# Autodesk Inventor assembly: A1-18002-100-00 Line boring skid
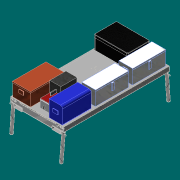
[picture p0: Inventor's stored thumbnail of the model, 180x180]
Saved by Autodesk Inventor 2017 (Build 210142000, 142)
## iProperties
Created: 2018-01-23
Part Number: A1-18002-100-00 Line boring skid
Document SubType Name: Assembly
Designer: Graeme_Van_Dongen
Mass: 2.94826e+06 g
Surface Area: 313203 cm^2
Volume: 587682 cm^3
Density: 5.01675 g/cm^3
Author: Graeme_Van_Dongen
## Documents named in this file (43)
- N:\A1 - Projects\A1-18\A1-18002--Alco Line boring skid\A1-18002-100-00 Line boring skid.iam
- N:\A1 - Projects\A1-18\A1-18002--Alco Line boring skid\Aluminum tool box.ipt
- N:\A1 - Projects\A1-18\A1-18002--Alco Line boring skid\Blue tool box.ipt
- N:\A1 - Projects\A1-18\A1-18002--Alco Line boring skid\Jobox tool box.ipt
- N:\A1 - Projects\A1-18\A1-18002--Alco Line boring skid\Pelican case.ipt
- N:\A1 - Projects\A1-18\A1-18002--Alco Line boring skid\2.25 bar x 8ft.ipt
- N:\A1 - Projects\A1-18\A1-18002--Alco Line boring skid\2.25 bar x 7ft.ipt
- N:\A1 - Projects\A1-18\A1-18002--Alco Line boring skid\2.25 bar x 5ft.ipt
- N:\A1 - Projects\A1-18\A1-18002--Alco Line boring skid\2.25 bar x 3.5ft.ipt
- N:\A1 - Projects\A1-18\A1-18002--Alco Line boring skid\2.25 bar x 3.25ft.ipt
- N:\A1 - Projects\A1-18\A1-18002--Alco Line boring skid\2.25 bar x 3ft.ipt
- N:\A1 - Projects\A1-18\A1-18002--Alco Line boring skid\1.25 bar x 4ft.ipt
- N:\A1 - Projects\A1-18\A1-18002--Alco Line boring skid\1.25 bar x 3ft.ipt
- N:\A1 - Projects\A1-18\A1-18002--Alco Line boring skid\1.25 bar x 2ft.ipt
- N:\A1 - Projects\A1-18\A1-18002--Alco Line boring skid\Welder.ipt
- N:\A1 - Projects\A1-18\A1-18002--Alco Line boring skid\A1-18002-100-20 2.25in x 8ft bar tube.ipt
- N:\A1 - Projects\A1-18\A1-18002--Alco Line boring skid\A1-18002-100-30 2.5in pipe cap.ipt
- ASME B16.11 Cap - Class 3000 2 1/2.ipt
- N:\A1 - Projects\A1-18\A1-18002--Alco Line boring skid\A1-18002-300-00 2.25in bar tube cap.iam
- N:\A1 - Projects\A1-18\A1-18002--Alco Line boring skid\A1-18002-100-21 2.25in x 7ft bar tube.ipt
- N:\A1 - Projects\A1-18\A1-18002--Alco Line boring skid\A1-18002-100-22 2.25in x 5ft bar tube.ipt
- N:\A1 - Projects\A1-18\A1-18002--Alco Line boring skid\A1-18002-100-23 2.25in x 3.5ft bar tube.ipt
- N:\A1 - Projects\A1-18\A1-18002--Alco Line boring skid\A1-18002-100-24 2.25in x 3.25ft bar tube.ipt
- N:\A1 - Projects\A1-18\A1-18002--Alco Line boring skid\A1-18002-100-25 2.25in x 3ft bar tube.ipt
- N:\A1 - Projects\A1-18\A1-18002--Alco Line boring skid\A1-18002-100-31 1.25in x 4ft bar tube.ipt
- N:\A1 - Projects\A1-18\A1-18002--Alco Line boring skid\A1-18002-100-32 1.25in x 3ft bar tube.ipt
- N:\A1 - Projects\A1-18\A1-18002--Alco Line boring skid\A1-18002-100-33 1.25in x 2ft bar tube.ipt
- N:\A1 - Projects\A1-18\A1-18002--Alco Line boring skid\A1-18002-100-36 1.5in pipe cap.ipt
- N:\A1 - Projects\A1-18\A1-18002--Alco Line boring skid\A1-18002-400-00 1.25in bar tube cap.iam
- N:\A1 - Projects\A1-18\A1-18002--Alco Line boring skid\Base frame skeleton.ipt
- N:\A1 - Projects\A1-18\A1-18002--Alco Line boring skid\A1-18002-200-00 Skid leg.iam
- N:\A1 - Projects\A1-18\A1-18002--Alco Line boring skid\Spring latch.ipt
- N:\A1 - Projects\A1-18\A1-18002--Alco Line boring skid\Weld-on hinge #218-109.ipt
- N:\A1 - Projects\A1-18\A1-18002--Alco Line boring skid\A1-18002-100-40 Pocket door plate.ipt
- N:\Inventor\Content Center Files\R2017\en-US\ANSI L(1)\AISC - L 1 x 1 x 1_8 - 32.ipt
- N:\A1 - Projects\A1-18\A1-18002--Alco Line boring skid\A1-18002-150-00 Line boring skid weldment.iam
- N:\Inventor\Content Center Files\R2017\en-US\MS 16624 (3100)\MS 16624 - 0.500S 3100.ipt
- N:\A1 - Projects\A1-18\A1-18002--Alco Line boring skid\Quick release pin.ipt
- N:\A1 - Projects\A1-18\A1-18002--Alco Line boring skid\A1-18002-100-50 Tube cradle - 2.875in.ipt
- N:\A1 - Projects\A1-18\A1-18002--Alco Line boring skid\A1-18002-100-51 Tube cradle - 1.900in.ipt
- N:\A1 - Projects\A1-18\A1-18002--Alco Line boring skid\A1-18002-100-53 Tube stop.ipt
- N:\A1 - Projects\A1-18\A1-18002--Alco Line boring skid\A1-18002-100-52 Tube stop.ipt
- N:\A1 - Projects\A1-18\A1-18002--Alco Line boring skid\A1-18002-100-54 Tube stop.ipt
## Components (101 placed, 41 different names)
1. A1-18002-150-00 Line boring skid weldment:1 [sub-assembly] — Flush:7, Flush:8, Flush:9, Mate:1, Mate:2, Mate:3, Mate:4, Mate:5, Angle:1, Angle:2, Angle:3, Angle:4, Angle:5, Mate:6, Angle:6, Mate:7, Mate:8, Mate:9, Angle:7, Mate:10, Mate:11, Mate:12, Mate:13, Mate:14, Mate:15, Mate:16, Mate:17, Mate:18, Flush:30, Flush:31, Flush:32, Flush:40, Insert:31, Angle:8, Insert:32, Angle:9, Insert:33, Insert:34, Angle:10, Tangent:42, Tangent:43, Angle:12, Angle:13, Angle:14, Angle:15, Angle:16, Angle:17, Angle:18, Angle:19, Angle:20, Angle:21, Angle:22, Angle:23, Angle:24, Angle:25, Angle:26, Angle:27, Angle:28, Angle:29, Angle:30, Angle:31, Angle:32, Angle:33, Angle:34, Angle:35, Angle:36, Angle:37, Mate:49, Mate:50, Mate:52, Mate:54, Mate:57, Mate:59, Mate:61, Mate:63, Mate:66, Mate:69, Mate:72
2. Base frame skeleton:1 — Flush:30, Flush:31, Flush:32
3. Aluminum tool box:1 — Mate:1, Angle:1, Flush:28, Flush:29
4. Aluminum tool box:2 — Mate:2, Angle:2, Flush:28
5. Blue tool box:1 — Mate:3, Angle:3, Flush:29
6. Jobox tool box:1 — Mate:4, Angle:4
7. Pelican case:1 — Mate:5, Angle:5
8. Welder:1 — Mate:6, Angle:6
9. A1-18002-100-40 Pocket door plate:1 — Mate:47, Flush:40, Mate:26, Mate:28, Mate:43, Mate:44, Flush:45, Mate:45, Flush:46, Flush:47, Flush:48, Flush:49, Angle:12
10. Spring latch:1 — Mate:26, Mate:28, Flush:41, Mate:48, Flush:48
11. Spring latch:2 — Flush:41, Mate:48, Flush:49
12. Weld-on hinge #218-109:1 — Flush:42, Mate:43, Tangent:42, Mate:46, Flush:47
13. Weld-on hinge #218-109:2 — Flush:42, Mate:46, Mate:47, Flush:46, Tangent:43
14. ANSI L (Equal angles) L 1 x 1 x 1/8 - 32:1 — Mate:44, Flush:45, Mate:45
15. A1-18002-100-20 2.25in x 8ft bar tube:1 — Insert:1, Insert:2, Mate:7, Angle:7, Flush:10, Flush:18
16. A1-18002-300-00 2.25in bar tube cap:1 [sub-assembly] — Insert:1, Mate:8, Mate:9, Insert:39
17. A1-18002-100-30 2.5in pipe cap:2 — Insert:2, Insert:19, Insert:37, Insert:38
18. A1-18002-100-21 2.25in x 7ft bar tube:1 — Insert:3, Insert:8, Flush:10, Flush:11, Flush:18, Flush:19
19. A1-18002-300-00 2.25in bar tube cap:2 [sub-assembly] — Insert:3, Mate:10, Insert:42
20. A1-18002-100-30 2.5in pipe cap:3 — Insert:8, Insert:20, Insert:40, Insert:41, Mate:51
21. A1-18002-100-22 2.25in x 5ft bar tube:1 — Insert:4, Insert:9, Flush:11, Flush:19, Flush:26, Flush:27
22. A1-18002-300-00 2.25in bar tube cap:3 [sub-assembly] — Insert:4, Mate:11, Insert:45
23. A1-18002-100-30 2.5in pipe cap:4 — Insert:9, Insert:21, Insert:43, Insert:44, Mate:53
24. A1-18002-100-22 2.25in x 5ft bar tube:2 — Insert:28, Insert:30, Flush:26, Flush:27, Flush:20, Flush:12
25. A1-18002-300-00 2.25in bar tube cap:7 [sub-assembly] — Insert:28, Mate:18, Insert:48
26. A1-18002-100-30 2.5in pipe cap:8 — Insert:29, Insert:30, Insert:46, Insert:47, Mate:56
27. A1-18002-100-23 2.25in x 3.5ft bar tube:1 — Insert:5, Insert:10, Flush:12, Flush:13, Flush:20, Flush:21
28. A1-18002-300-00 2.25in bar tube cap:4 [sub-assembly] — Insert:5, Mate:12, Insert:50
29. A1-18002-100-30 2.5in pipe cap:5 — Insert:10, Insert:22, Insert:49, Mate:58
30. A1-18002-100-24 2.25in x 3.25ft bar tube:1 — Insert:6, Insert:11, Flush:13, Flush:14, Flush:21, Flush:22
31. A1-18002-300-00 2.25in bar tube cap:5 [sub-assembly] — Insert:6, Mate:13, Insert:52
32. A1-18002-100-30 2.5in pipe cap:6 — Insert:11, Insert:23, Insert:51, Mate:60
33. A1-18002-100-25 2.25in x 3ft bar tube:1 — Insert:7, Insert:12, Flush:14, Flush:15, Flush:22, Flush:23
34. A1-18002-300-00 2.25in bar tube cap:6 [sub-assembly] — Insert:7, Mate:14, Insert:54
35. A1-18002-100-30 2.5in pipe cap:7 — Insert:12, Insert:24, Insert:53, Mate:62
36. A1-18002-100-31 1.25in x 4ft bar tube:1 — Insert:13, Insert:16, Flush:15, Flush:16, Flush:23, Flush:24
37. A1-18002-400-00 1.25in bar tube cap:1 [sub-assembly] — Insert:13, Mate:15, Insert:57
38. A1-18002-100-36 1.5in pipe cap:1 — Insert:16, Insert:25, Insert:55, Insert:56, Mate:65
39. A1-18002-100-32 1.25in x 3ft bar tube:1 — Insert:14, Insert:17, Flush:16, Flush:17, Flush:24, Flush:25
40. A1-18002-400-00 1.25in bar tube cap:2 [sub-assembly] — Insert:14, Mate:16, Insert:59
41. A1-18002-100-36 1.5in pipe cap:2 — Insert:17, Insert:26, Insert:58, Mate:68
42. A1-18002-100-33 1.25in x 2ft bar tube:1 — Insert:15, Insert:18, Flush:17, Flush:25
43. A1-18002-400-00 1.25in bar tube cap:3 [sub-assembly] — Insert:15, Mate:17, Insert:61
44. A1-18002-100-36 1.5in pipe cap:3 — Insert:18, Insert:27, Insert:60, Mate:71
45. 2.25 bar x 8ft:1 — Insert:19
46. 2.25 bar x 7ft:1 — Insert:20
47. 2.25 bar x 5ft:1 — Insert:29
48. 2.25 bar x 5ft:2 — Insert:21
49. 2.25 bar x 3.5ft:1 — Insert:22
50. 2.25 bar x 3.25ft:1 — Insert:23
51. 2.25 bar x 3ft:1 — Insert:24
52. 1.25 bar x 4ft:1 — Insert:25
53. 1.25 bar x 3ft:1 — Insert:26
54. 1.25 bar x 2ft:1 — Insert:27
55. A1-18002-100-50 Tube cradle - 2.875in:1 — Insert:37, Angle:13, Flush:50
56. A1-18002-100-50 Tube cradle - 2.875in:2 — Insert:38, Angle:14
57. A1-18002-100-50 Tube cradle - 2.875in:3 — Insert:39, Angle:15
58. A1-18002-100-50 Tube cradle - 2.875in:4 — Insert:40, Angle:16, Flush:51
59. A1-18002-100-50 Tube cradle - 2.875in:5 — Insert:41, Angle:17
60. A1-18002-100-50 Tube cradle - 2.875in:6 — Insert:42, Angle:18
61. A1-18002-100-50 Tube cradle - 2.875in:7 — Insert:43, Angle:19, Flush:52
62. A1-18002-100-50 Tube cradle - 2.875in:8 — Insert:44, Angle:20
63. A1-18002-100-50 Tube cradle - 2.875in:9 — Insert:45, Angle:21
64. A1-18002-100-50 Tube cradle - 2.875in:10 — Insert:46, Angle:22, Flush:56
65. A1-18002-100-50 Tube cradle - 2.875in:11 — Insert:47, Angle:23
66. A1-18002-100-50 Tube cradle - 2.875in:12 — Insert:48, Angle:24
67. A1-18002-100-50 Tube cradle - 2.875in:13 — Insert:49, Angle:25, Flush:57
68. A1-18002-100-50 Tube cradle - 2.875in:14 — Insert:50, Angle:26
69. A1-18002-100-50 Tube cradle - 2.875in:15 — Insert:51, Angle:27, Flush:58
70. A1-18002-100-50 Tube cradle - 2.875in:16 — Insert:52, Angle:28
71. A1-18002-100-50 Tube cradle - 2.875in:17 — Insert:53, Angle:29, Flush:59
72. A1-18002-100-50 Tube cradle - 2.875in:18 — Insert:54, Angle:30
73. A1-18002-100-51 Tube cradle - 1.900in:1 — Insert:55, Angle:31, Mate:64
74. A1-18002-100-51 Tube cradle - 1.900in:2 — Insert:56, Angle:32
75. A1-18002-100-51 Tube cradle - 1.900in:3 — Insert:57, Angle:33
76. A1-18002-100-51 Tube cradle - 1.900in:4 — Insert:58, Angle:34, Mate:67
77. A1-18002-100-51 Tube cradle - 1.900in:5 — Insert:59, Angle:35
78. A1-18002-100-51 Tube cradle - 1.900in:6 — Insert:60, Angle:36, Mate:70
79. A1-18002-100-51 Tube cradle - 1.900in:7 — Insert:61, Angle:37
80. A1-18002-100-53 Tube stop:1 — Flush:50, Mate:49, Mate:50
81. A1-18002-100-52 Tube stop:1 — Flush:51, Mate:51, Mate:52
82. A1-18002-100-52 Tube stop:2 — Flush:52, Mate:53, Mate:54
83. A1-18002-100-52 Tube stop:3 — Flush:56, Mate:56, Mate:57
84. A1-18002-100-52 Tube stop:4 — Flush:57, Mate:58, Mate:59
85. A1-18002-100-52 Tube stop:5 — Flush:58, Mate:60, Mate:61
86. A1-18002-100-52 Tube stop:6 — Flush:59, Mate:62, Mate:63
87. A1-18002-100-54 Tube stop:1 — Mate:64, Mate:65, Mate:66
88. A1-18002-100-54 Tube stop:2 — Mate:67, Mate:68, Mate:69
89. A1-18002-100-54 Tube stop:3 — Mate:70, Mate:71, Mate:72
90. A1-18002-200-00 Skid leg:1 [sub-assembly] — Insert:31, Angle:8, Insert:35
91. A1-18002-200-00 Skid leg:2 [sub-assembly] — Insert:32, Angle:9, Insert:36
92. Industrial External Retaining Rings, Series 3100 0.500:1 — Insert:33
93. Industrial External Retaining Rings, Series 3100 0.500:2 — Insert:34
94. Quick release pin:1 — Insert:35, Angle:10, Angle:11
95. Quick release pin:2 — Insert:36, Angle:11
96. A1-18002-200-00 Skid leg:3 [sub-assembly]
97. A1-18002-200-00 Skid leg:4 [sub-assembly]
98. Industrial External Retaining Rings, Series 3100 0.500:3
99. Industrial External Retaining Rings, Series 3100 0.500:4
100. Quick release pin:3
101. Quick release pin:4
## Component patterns: (2 elements, first: A1-18002-200-00 Skid leg:1 + A1-18002-200-00 Skid leg:2 + Industrial External Retaining Rings, Series 3100 0.500:1 + Industrial External Retaining Rings, Series 3100 0.500:2 + Quick release pin:1 + Quick release pin:2)
## Relationships (190: Insert 61, Mate 49, Flush 41, Angle 37, Tangent 2)
- Flush:7: A1-18002-150-00 Line boring skid weldment:1
- Flush:8: A1-18002-150-00 Line boring skid weldment:1
- Flush:9: A1-18002-150-00 Line boring skid weldment:1
- Mate:1: A1-18002-150-00 Line boring skid weldment:1 ↔ Aluminum tool box:1
- Mate:2: A1-18002-150-00 Line boring skid weldment:1 ↔ Aluminum tool box:2
- Mate:3: A1-18002-150-00 Line boring skid weldment:1 ↔ Blue tool box:1
- Mate:4: A1-18002-150-00 Line boring skid weldment:1 ↔ Jobox tool box:1
- Mate:5: A1-18002-150-00 Line boring skid weldment:1 ↔ Pelican case:1
- Angle:1 (0 deg): A1-18002-150-00 Line boring skid weldment:1 ↔ Aluminum tool box:1
- Angle:2 (0 deg): A1-18002-150-00 Line boring skid weldment:1 ↔ Aluminum tool box:2
- Angle:3 (0 deg): A1-18002-150-00 Line boring skid weldment:1 ↔ Blue tool box:1
- Angle:4 (180 deg): A1-18002-150-00 Line boring skid weldment:1 ↔ Jobox tool box:1
- Angle:5 (180 deg): A1-18002-150-00 Line boring skid weldment:1 ↔ Pelican case:1
- Mate:6: A1-18002-150-00 Line boring skid weldment:1 ↔ Welder:1
- Angle:6 (0 deg): A1-18002-150-00 Line boring skid weldment:1 ↔ Welder:1
- Insert:1: A1-18002-100-20 2.25in x 8ft bar tube:1 ↔ A1-18002-300-00 2.25in bar tube cap:1
- Insert:2: A1-18002-100-20 2.25in x 8ft bar tube:1 ↔ A1-18002-100-30 2.5in pipe cap:2
- Insert:3: A1-18002-100-21 2.25in x 7ft bar tube:1 ↔ A1-18002-300-00 2.25in bar tube cap:2
- Insert:4: A1-18002-100-22 2.25in x 5ft bar tube:1 ↔ A1-18002-300-00 2.25in bar tube cap:3
- Insert:5: A1-18002-100-23 2.25in x 3.5ft bar tube:1 ↔ A1-18002-300-00 2.25in bar tube cap:4
- Insert:6: A1-18002-100-24 2.25in x 3.25ft bar tube:1 ↔ A1-18002-300-00 2.25in bar tube cap:5
- Insert:7: A1-18002-100-25 2.25in x 3ft bar tube:1 ↔ A1-18002-300-00 2.25in bar tube cap:6
- Insert:8: A1-18002-100-21 2.25in x 7ft bar tube:1 ↔ A1-18002-100-30 2.5in pipe cap:3
- Insert:9: A1-18002-100-22 2.25in x 5ft bar tube:1 ↔ A1-18002-100-30 2.5in pipe cap:4
- Insert:10: A1-18002-100-23 2.25in x 3.5ft bar tube:1 ↔ A1-18002-100-30 2.5in pipe cap:5
- Insert:11: A1-18002-100-24 2.25in x 3.25ft bar tube:1 ↔ A1-18002-100-30 2.5in pipe cap:6
- Insert:12: A1-18002-100-25 2.25in x 3ft bar tube:1 ↔ A1-18002-100-30 2.5in pipe cap:7
- Insert:13: A1-18002-100-31 1.25in x 4ft bar tube:1 ↔ A1-18002-400-00 1.25in bar tube cap:1
- Insert:14: A1-18002-100-32 1.25in x 3ft bar tube:1 ↔ A1-18002-400-00 1.25in bar tube cap:2
- Insert:15: A1-18002-100-33 1.25in x 2ft bar tube:1 ↔ A1-18002-400-00 1.25in bar tube cap:3
- Insert:16: A1-18002-100-31 1.25in x 4ft bar tube:1 ↔ A1-18002-100-36 1.5in pipe cap:1
- Insert:17: A1-18002-100-32 1.25in x 3ft bar tube:1 ↔ A1-18002-100-36 1.5in pipe cap:2
- Insert:18: A1-18002-100-33 1.25in x 2ft bar tube:1 ↔ A1-18002-100-36 1.5in pipe cap:3
- Mate:7 (50.8 mm): A1-18002-150-00 Line boring skid weldment:1 ↔ A1-18002-100-20 2.25in x 8ft bar tube:1
- Mate:8 (-46.0375 mm): A1-18002-150-00 Line boring skid weldment:1 ↔ A1-18002-300-00 2.25in bar tube cap:1
- Mate:9 (-88.9 mm): A1-18002-150-00 Line boring skid weldment:1 ↔ A1-18002-300-00 2.25in bar tube cap:1
- Angle:7 (-15 deg): A1-18002-150-00 Line boring skid weldment:1 ↔ A1-18002-100-20 2.25in x 8ft bar tube:1
- Flush:10: A1-18002-100-20 2.25in x 8ft bar tube:1 ↔ A1-18002-100-21 2.25in x 7ft bar tube:1
- Flush:11: A1-18002-100-21 2.25in x 7ft bar tube:1 ↔ A1-18002-100-22 2.25in x 5ft bar tube:1
- Flush:12: A1-18002-100-22 2.25in x 5ft bar tube:2 ↔ A1-18002-100-23 2.25in x 3.5ft bar tube:1
- Flush:13: A1-18002-100-23 2.25in x 3.5ft bar tube:1 ↔ A1-18002-100-24 2.25in x 3.25ft bar tube:1
- Flush:14: A1-18002-100-24 2.25in x 3.25ft bar tube:1 ↔ A1-18002-100-25 2.25in x 3ft bar tube:1
- Flush:15: A1-18002-100-25 2.25in x 3ft bar tube:1 ↔ A1-18002-100-31 1.25in x 4ft bar tube:1
- Flush:16: A1-18002-100-31 1.25in x 4ft bar tube:1 ↔ A1-18002-100-32 1.25in x 3ft bar tube:1
- Flush:17: A1-18002-100-32 1.25in x 3ft bar tube:1 ↔ A1-18002-100-33 1.25in x 2ft bar tube:1
- Flush:18 (107.95 mm): A1-18002-100-20 2.25in x 8ft bar tube:1 ↔ A1-18002-100-21 2.25in x 7ft bar tube:1
- Flush:19 (107.95 mm): A1-18002-100-21 2.25in x 7ft bar tube:1 ↔ A1-18002-100-22 2.25in x 5ft bar tube:1
- Flush:20 (107.95 mm): A1-18002-100-22 2.25in x 5ft bar tube:2 ↔ A1-18002-100-23 2.25in x 3.5ft bar tube:1
- Flush:21 (107.95 mm): A1-18002-100-23 2.25in x 3.5ft bar tube:1 ↔ A1-18002-100-24 2.25in x 3.25ft bar tube:1
- Flush:22 (107.95 mm): A1-18002-100-24 2.25in x 3.25ft bar tube:1 ↔ A1-18002-100-25 2.25in x 3ft bar tube:1
- Flush:23 (93.6625 mm): A1-18002-100-25 2.25in x 3ft bar tube:1 ↔ A1-18002-100-31 1.25in x 4ft bar tube:1
- Flush:24 (79.375 mm): A1-18002-100-31 1.25in x 4ft bar tube:1 ↔ A1-18002-100-32 1.25in x 3ft bar tube:1
- Flush:25 (79.375 mm): A1-18002-100-32 1.25in x 3ft bar tube:1 ↔ A1-18002-100-33 1.25in x 2ft bar tube:1
- Mate:10 (-46.0375 mm): A1-18002-150-00 Line boring skid weldment:1 ↔ A1-18002-300-00 2.25in bar tube cap:2
- Mate:11 (-46.0375 mm): A1-18002-150-00 Line boring skid weldment:1 ↔ A1-18002-300-00 2.25in bar tube cap:3
- Mate:12 (-46.0375 mm): A1-18002-150-00 Line boring skid weldment:1 ↔ A1-18002-300-00 2.25in bar tube cap:4
- Mate:13 (-46.0375 mm): A1-18002-150-00 Line boring skid weldment:1 ↔ A1-18002-300-00 2.25in bar tube cap:5
- Mate:14 (-46.0375 mm): A1-18002-150-00 Line boring skid weldment:1 ↔ A1-18002-300-00 2.25in bar tube cap:6
- Mate:15 (-42.0688 mm): A1-18002-150-00 Line boring skid weldment:1 ↔ A1-18002-400-00 1.25in bar tube cap:1
- Mate:16 (-42.0688 mm): A1-18002-150-00 Line boring skid weldment:1 ↔ A1-18002-400-00 1.25in bar tube cap:2
- Mate:17 (-42.0688 mm): A1-18002-150-00 Line boring skid weldment:1 ↔ A1-18002-400-00 1.25in bar tube cap:3
- Insert:19: A1-18002-100-30 2.5in pipe cap:2 ↔ 2.25 bar x 8ft:1
- Insert:20: A1-18002-100-30 2.5in pipe cap:3 ↔ 2.25 bar x 7ft:1
- Insert:21: A1-18002-100-30 2.5in pipe cap:4 ↔ 2.25 bar x 5ft:2
- Insert:22: A1-18002-100-30 2.5in pipe cap:5 ↔ 2.25 bar x 3.5ft:1
- Insert:23: A1-18002-100-30 2.5in pipe cap:6 ↔ 2.25 bar x 3.25ft:1
- Insert:24: A1-18002-100-30 2.5in pipe cap:7 ↔ 2.25 bar x 3ft:1
- Insert:25: A1-18002-100-36 1.5in pipe cap:1 ↔ 1.25 bar x 4ft:1
- Insert:26: A1-18002-100-36 1.5in pipe cap:2 ↔ 1.25 bar x 3ft:1
- Insert:27: A1-18002-100-36 1.5in pipe cap:3 ↔ 1.25 bar x 2ft:1
- Insert:28: A1-18002-100-22 2.25in x 5ft bar tube:2 ↔ A1-18002-300-00 2.25in bar tube cap:7
- Insert:29: A1-18002-100-30 2.5in pipe cap:8 ↔ 2.25 bar x 5ft:1
- Insert:30: A1-18002-100-22 2.25in x 5ft bar tube:2 ↔ A1-18002-100-30 2.5in pipe cap:8
- Flush:26 (107.95 mm): A1-18002-100-22 2.25in x 5ft bar tube:1 ↔ A1-18002-100-22 2.25in x 5ft bar tube:2
- Mate:18 (-46.0375 mm): A1-18002-150-00 Line boring skid weldment:1 ↔ A1-18002-300-00 2.25in bar tube cap:7
- Flush:27: A1-18002-100-22 2.25in x 5ft bar tube:1 ↔ A1-18002-100-22 2.25in x 5ft bar tube:2
- Flush:28: Aluminum tool box:1 ↔ Aluminum tool box:2
- Flush:29: Aluminum tool box:1 ↔ Blue tool box:1
- Flush:30: A1-18002-150-00 Line boring skid weldment:1 ↔ Base frame skeleton:1
- Flush:31: A1-18002-150-00 Line boring skid weldment:1 ↔ Base frame skeleton:1
- Flush:32 (101.6 mm): A1-18002-150-00 Line boring skid weldment:1 ↔ Base frame skeleton:1
- Mate:47: A1-18002-100-40 Pocket door plate:1 ↔ Weld-on hinge #218-109:2
- Flush:40: A1-18002-150-00 Line boring skid weldment:1 ↔ A1-18002-100-40 Pocket door plate:1
- Mate:26: A1-18002-100-40 Pocket door plate:1 ↔ Spring latch:1
- Mate:28 (-12.7 mm): A1-18002-100-40 Pocket door plate:1 ↔ Spring latch:1
- Flush:41: Spring latch:1 ↔ Spring latch:2
- Flush:42: Weld-on hinge #218-109:1 ↔ Weld-on hinge #218-109:2
- Mate:43 (-5.0038 mm): A1-18002-100-40 Pocket door plate:1 ↔ Weld-on hinge #218-109:1
- Mate:44: A1-18002-100-40 Pocket door plate:1 ↔ ANSI L (Equal angles) L 1 x 1 x 1/8 - 32:1
- Flush:45 (22.225 mm): A1-18002-100-40 Pocket door plate:1 ↔ ANSI L (Equal angles) L 1 x 1 x 1/8 - 32:1
- Mate:45: A1-18002-100-40 Pocket door plate:1 ↔ ANSI L (Equal angles) L 1 x 1 x 1/8 - 32:1
- Insert:31: A1-18002-150-00 Line boring skid weldment:1 ↔ A1-18002-200-00 Skid leg:1
- Angle:8 (0 deg): A1-18002-150-00 Line boring skid weldment:1 ↔ A1-18002-200-00 Skid leg:1
- Insert:32: A1-18002-150-00 Line boring skid weldment:1 ↔ A1-18002-200-00 Skid leg:2
- Angle:9 (0 deg): A1-18002-150-00 Line boring skid weldment:1 ↔ A1-18002-200-00 Skid leg:2
- Insert:33: A1-18002-150-00 Line boring skid weldment:1 ↔ Industrial External Retaining Rings, Series 3100 0.500:1
- Insert:34: A1-18002-150-00 Line boring skid weldment:1 ↔ Industrial External Retaining Rings, Series 3100 0.500:2
- Insert:35: A1-18002-200-00 Skid leg:1 ↔ Quick release pin:1
- Angle:10 (0 deg): A1-18002-150-00 Line boring skid weldment:1 ↔ Quick release pin:1
- Insert:36: A1-18002-200-00 Skid leg:2 ↔ Quick release pin:2
- Angle:11 (0 deg): Quick release pin:1 ↔ Quick release pin:2
- Tangent:42: A1-18002-150-00 Line boring skid weldment:1 ↔ Weld-on hinge #218-109:1
- Mate:46: Weld-on hinge #218-109:1 ↔ Weld-on hinge #218-109:2
- Flush:46 (127 mm): A1-18002-100-40 Pocket door plate:1 ↔ Weld-on hinge #218-109:2
- Flush:47 (127 mm): A1-18002-100-40 Pocket door plate:1 ↔ Weld-on hinge #218-109:1
- Mate:48: Spring latch:1 ↔ Spring latch:2
- Flush:48 (10.3188 mm): A1-18002-100-40 Pocket door plate:1 ↔ Spring latch:1
- Flush:49 (10.3188 mm): A1-18002-100-40 Pocket door plate:1 ↔ Spring latch:2
- Tangent:43 (31.75 mm): A1-18002-150-00 Line boring skid weldment:1 ↔ Weld-on hinge #218-109:2
- Angle:12 (102.01 deg): A1-18002-150-00 Line boring skid weldment:1 ↔ A1-18002-100-40 Pocket door plate:1
- Insert:37: A1-18002-100-30 2.5in pipe cap:2 ↔ A1-18002-100-50 Tube cradle - 2.875in:1
- Angle:13 (0 deg): A1-18002-150-00 Line boring skid weldment:1 ↔ A1-18002-100-50 Tube cradle - 2.875in:1
- Insert:38 (1049.3375 mm): A1-18002-100-30 2.5in pipe cap:2 ↔ A1-18002-100-50 Tube cradle - 2.875in:2
- Angle:14 (0 deg): A1-18002-150-00 Line boring skid weldment:1 ↔ A1-18002-100-50 Tube cradle - 2.875in:2
- Insert:39: A1-18002-300-00 2.25in bar tube cap:1 ↔ A1-18002-100-50 Tube cradle - 2.875in:3
- Angle:15 (0 deg): A1-18002-150-00 Line boring skid weldment:1 ↔ A1-18002-100-50 Tube cradle - 2.875in:3
- Insert:40: A1-18002-100-30 2.5in pipe cap:3 ↔ A1-18002-100-50 Tube cradle - 2.875in:4
- Angle:16 (0 deg): A1-18002-150-00 Line boring skid weldment:1 ↔ A1-18002-100-50 Tube cradle - 2.875in:4
- Insert:41 (922.3375 mm): A1-18002-100-30 2.5in pipe cap:3 ↔ A1-18002-100-50 Tube cradle - 2.875in:5
- Angle:17 (0 deg): A1-18002-150-00 Line boring skid weldment:1 ↔ A1-18002-100-50 Tube cradle - 2.875in:5
- Insert:42: A1-18002-300-00 2.25in bar tube cap:2 ↔ A1-18002-100-50 Tube cradle - 2.875in:6
- Angle:18 (0 deg): A1-18002-150-00 Line boring skid weldment:1 ↔ A1-18002-100-50 Tube cradle - 2.875in:6
- Insert:43: A1-18002-100-30 2.5in pipe cap:4 ↔ A1-18002-100-50 Tube cradle - 2.875in:7
- Angle:19 (0 deg): A1-18002-150-00 Line boring skid weldment:1 ↔ A1-18002-100-50 Tube cradle - 2.875in:7
- Insert:44 (617.5375 mm): A1-18002-100-30 2.5in pipe cap:4 ↔ A1-18002-100-50 Tube cradle - 2.875in:8
- Angle:20 (0 deg): A1-18002-150-00 Line boring skid weldment:1 ↔ A1-18002-100-50 Tube cradle - 2.875in:8
- Insert:45: A1-18002-300-00 2.25in bar tube cap:3 ↔ A1-18002-100-50 Tube cradle - 2.875in:9
- Angle:21 (0 deg): A1-18002-150-00 Line boring skid weldment:1 ↔ A1-18002-100-50 Tube cradle - 2.875in:9
- Insert:46: A1-18002-100-30 2.5in pipe cap:8 ↔ A1-18002-100-50 Tube cradle - 2.875in:10
- Angle:22 (0 deg): A1-18002-150-00 Line boring skid weldment:1 ↔ A1-18002-100-50 Tube cradle - 2.875in:10
- Insert:47 (617.5375 mm): A1-18002-100-30 2.5in pipe cap:8 ↔ A1-18002-100-50 Tube cradle - 2.875in:11
- Angle:23 (0 deg): A1-18002-150-00 Line boring skid weldment:1 ↔ A1-18002-100-50 Tube cradle - 2.875in:11
- Insert:48: A1-18002-300-00 2.25in bar tube cap:7 ↔ A1-18002-100-50 Tube cradle - 2.875in:12
- Angle:24 (0 deg): A1-18002-150-00 Line boring skid weldment:1 ↔ A1-18002-100-50 Tube cradle - 2.875in:12
- Insert:49: A1-18002-100-30 2.5in pipe cap:5 ↔ A1-18002-100-50 Tube cradle - 2.875in:13
- Angle:25 (0 deg): A1-18002-150-00 Line boring skid weldment:1 ↔ A1-18002-100-50 Tube cradle - 2.875in:13
- Insert:50: A1-18002-300-00 2.25in bar tube cap:4 ↔ A1-18002-100-50 Tube cradle - 2.875in:14
- Angle:26 (0 deg): A1-18002-150-00 Line boring skid weldment:1 ↔ A1-18002-100-50 Tube cradle - 2.875in:14
- Insert:51: A1-18002-100-30 2.5in pipe cap:6 ↔ A1-18002-100-50 Tube cradle - 2.875in:15
- Angle:27 (0 deg): A1-18002-150-00 Line boring skid weldment:1 ↔ A1-18002-100-50 Tube cradle - 2.875in:15
- Insert:52: A1-18002-300-00 2.25in bar tube cap:5 ↔ A1-18002-100-50 Tube cradle - 2.875in:16
- Angle:28 (0 deg): A1-18002-150-00 Line boring skid weldment:1 ↔ A1-18002-100-50 Tube cradle - 2.875in:16
- Insert:53: A1-18002-100-30 2.5in pipe cap:7 ↔ A1-18002-100-50 Tube cradle - 2.875in:17
- Angle:29 (0 deg): A1-18002-150-00 Line boring skid weldment:1 ↔ A1-18002-100-50 Tube cradle - 2.875in:17
- Insert:54: A1-18002-300-00 2.25in bar tube cap:6 ↔ A1-18002-100-50 Tube cradle - 2.875in:18
- Angle:30 (0 deg): A1-18002-150-00 Line boring skid weldment:1 ↔ A1-18002-100-50 Tube cradle - 2.875in:18
- Insert:55: A1-18002-100-36 1.5in pipe cap:1 ↔ A1-18002-100-51 Tube cradle - 1.900in:1
- Angle:31 (0 deg): A1-18002-150-00 Line boring skid weldment:1 ↔ A1-18002-100-51 Tube cradle - 1.900in:1
- Insert:56 (466.725 mm): A1-18002-100-36 1.5in pipe cap:1 ↔ A1-18002-100-51 Tube cradle - 1.900in:2
- Angle:32 (0 deg): A1-18002-150-00 Line boring skid weldment:1 ↔ A1-18002-100-51 Tube cradle - 1.900in:2
- Insert:57: A1-18002-400-00 1.25in bar tube cap:1 ↔ A1-18002-100-51 Tube cradle - 1.900in:3
- Angle:33 (0 deg): A1-18002-150-00 Line boring skid weldment:1 ↔ A1-18002-100-51 Tube cradle - 1.900in:3
- Insert:58: A1-18002-100-36 1.5in pipe cap:2 ↔ A1-18002-100-51 Tube cradle - 1.900in:4
- Angle:34 (0 deg): A1-18002-150-00 Line boring skid weldment:1 ↔ A1-18002-100-51 Tube cradle - 1.900in:4
- Insert:59: A1-18002-400-00 1.25in bar tube cap:2 ↔ A1-18002-100-51 Tube cradle - 1.900in:5
- Angle:35 (0 deg): A1-18002-150-00 Line boring skid weldment:1 ↔ A1-18002-100-51 Tube cradle - 1.900in:5
- Insert:60: A1-18002-100-36 1.5in pipe cap:3 ↔ A1-18002-100-51 Tube cradle - 1.900in:6
- Angle:36 (0 deg): A1-18002-150-00 Line boring skid weldment:1 ↔ A1-18002-100-51 Tube cradle - 1.900in:6
- Insert:61: A1-18002-400-00 1.25in bar tube cap:3 ↔ A1-18002-100-51 Tube cradle - 1.900in:7
- Angle:37 (0 deg): A1-18002-150-00 Line boring skid weldment:1 ↔ A1-18002-100-51 Tube cradle - 1.900in:7
- Flush:50: A1-18002-100-50 Tube cradle - 2.875in:1 ↔ A1-18002-100-53 Tube stop:1
- Mate:49 (15.875 mm): A1-18002-150-00 Line boring skid weldment:1 ↔ A1-18002-100-53 Tube stop:1
- Mate:50: A1-18002-150-00 Line boring skid weldment:1 ↔ A1-18002-100-53 Tube stop:1
- Flush:51: A1-18002-100-50 Tube cradle - 2.875in:4 ↔ A1-18002-100-52 Tube stop:1
- Mate:51: A1-18002-100-30 2.5in pipe cap:3 ↔ A1-18002-100-52 Tube stop:1
- Mate:52: A1-18002-150-00 Line boring skid weldment:1 ↔ A1-18002-100-52 Tube stop:1
- Flush:52: A1-18002-100-50 Tube cradle - 2.875in:7 ↔ A1-18002-100-52 Tube stop:2
- Mate:53: A1-18002-100-30 2.5in pipe cap:4 ↔ A1-18002-100-52 Tube stop:2
- Mate:54: A1-18002-150-00 Line boring skid weldment:1 ↔ A1-18002-100-52 Tube stop:2
- Flush:56: A1-18002-100-50 Tube cradle - 2.875in:10 ↔ A1-18002-100-52 Tube stop:3
- Mate:56: A1-18002-100-30 2.5in pipe cap:8 ↔ A1-18002-100-52 Tube stop:3
- Mate:57: A1-18002-150-00 Line boring skid weldment:1 ↔ A1-18002-100-52 Tube stop:3
- Flush:57: A1-18002-100-50 Tube cradle - 2.875in:13 ↔ A1-18002-100-52 Tube stop:4
- Mate:58: A1-18002-100-30 2.5in pipe cap:5 ↔ A1-18002-100-52 Tube stop:4
- Mate:59: A1-18002-150-00 Line boring skid weldment:1 ↔ A1-18002-100-52 Tube stop:4
- Flush:58: A1-18002-100-50 Tube cradle - 2.875in:15 ↔ A1-18002-100-52 Tube stop:5
- Mate:60: A1-18002-100-30 2.5in pipe cap:6 ↔ A1-18002-100-52 Tube stop:5
- Mate:61: A1-18002-150-00 Line boring skid weldment:1 ↔ A1-18002-100-52 Tube stop:5
- Flush:59: A1-18002-100-50 Tube cradle - 2.875in:17 ↔ A1-18002-100-52 Tube stop:6
- Mate:62: A1-18002-100-30 2.5in pipe cap:7 ↔ A1-18002-100-52 Tube stop:6
- Mate:63: A1-18002-150-00 Line boring skid weldment:1 ↔ A1-18002-100-52 Tube stop:6
- Mate:64: A1-18002-100-51 Tube cradle - 1.900in:1 ↔ A1-18002-100-54 Tube stop:1
- Mate:65: A1-18002-100-36 1.5in pipe cap:1 ↔ A1-18002-100-54 Tube stop:1
- Mate:66: A1-18002-150-00 Line boring skid weldment:1 ↔ A1-18002-100-54 Tube stop:1
- Mate:67: A1-18002-100-51 Tube cradle - 1.900in:4 ↔ A1-18002-100-54 Tube stop:2
- Mate:68: A1-18002-100-36 1.5in pipe cap:2 ↔ A1-18002-100-54 Tube stop:2
- Mate:69: A1-18002-150-00 Line boring skid weldment:1 ↔ A1-18002-100-54 Tube stop:2
- Mate:70: A1-18002-100-51 Tube cradle - 1.900in:6 ↔ A1-18002-100-54 Tube stop:3
- Mate:71: A1-18002-100-36 1.5in pipe cap:3 ↔ A1-18002-100-54 Tube stop:3
- Mate:72: A1-18002-150-00 Line boring skid weldment:1 ↔ A1-18002-100-54 Tube stop:3
